# Autodesk Inventor assembly: vrRig_v01r1_bpFull
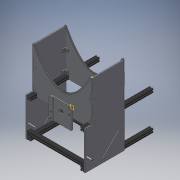
[picture p0: Inventor's stored thumbnail of the model, 180x180]
Saved by Autodesk Inventor 2016 (Build 200138000, 138)
## iProperties
Created: 2019-01-04
Part Number: vrRig_v01r1_bpFull
Document SubType Name: Assembly
Designer: harveylab
Author: harveylab
## Documents named in this file (3)
- C:\Users\harveylab\Documents\GitHub\HarVR\Hardware\BackProjection\vrRig_v01r1_bpFull.iam
- C:\Users\harveylab\Documents\GitHub\HarVR\Hardware\BackProjection\vrRig_v01r1_bpBox.iam
- C:\Users\harveylab\Documents\GitHub\HarVR\Hardware\BackProjection\TL_XE25L18_rail.ipt
## Components (5 placed, 2 different names)
1. vrRig_v01r1_bpBox:1 [sub-assembly] — Mate:1, Mate:2, Flush:1, Mate:3, Mate:4, Flush:2, Mate:5, Flush:3, Flush:4, Flush:5, Mate:6, Flush:6
2. TL_XE25L18_rail:1 — Mate:1, Mate:2, Flush:1
3. TL_XE25L18_rail:2 — Mate:3, Mate:4, Flush:2
4. TL_XE25L18_rail:3 — Mate:5, Flush:3, Flush:4
5. TL_XE25L18_rail:4 — Flush:5, Mate:6, Flush:6
## Relationships (12: Mate 6, Flush 6)
- Mate:1: vrRig_v01r1_bpBox:1 ↔ TL_XE25L18_rail:1
- Mate:2: vrRig_v01r1_bpBox:1 ↔ TL_XE25L18_rail:1
- Flush:1: vrRig_v01r1_bpBox:1 ↔ TL_XE25L18_rail:1
- Mate:3: vrRig_v01r1_bpBox:1 ↔ TL_XE25L18_rail:2
- Mate:4: vrRig_v01r1_bpBox:1 ↔ TL_XE25L18_rail:2
- Flush:2: vrRig_v01r1_bpBox:1 ↔ TL_XE25L18_rail:2
- Mate:5: vrRig_v01r1_bpBox:1 ↔ TL_XE25L18_rail:3
- Flush:3: vrRig_v01r1_bpBox:1 ↔ TL_XE25L18_rail:3
- Flush:4: vrRig_v01r1_bpBox:1 ↔ TL_XE25L18_rail:3
- Flush:5: vrRig_v01r1_bpBox:1 ↔ TL_XE25L18_rail:4
- Mate:6: vrRig_v01r1_bpBox:1 ↔ TL_XE25L18_rail:4
- Flush:6: vrRig_v01r1_bpBox:1 ↔ TL_XE25L18_rail:4
